# Autodesk Inventor assembly: 02EnsambleJarron
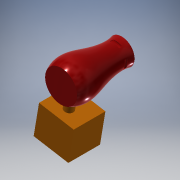
[picture p0: Inventor's stored thumbnail of the model, 180x180]
Saved by Autodesk Inventor 2018 (Build 220112000, 112)
## iProperties
Created: 2020-06-23
Part Number: 02EnsambleJarron
Document SubType Name: Assembly
Designer: Ivan
Author: Ivan
## Documents named in this file (3)
- C:\Users\Ivan\Documents\GitHub\Proyectos980\Modelos3D\02EnsambleJarron.iam
- C:\Users\Ivan\Documents\GitHub\Proyectos980\Modelos3D\02BombaJarron.ipt
- C:\Users\Ivan\Documents\GitHub\Proyectos980\Modelos3D\02Jarron.ipt
## Components (2 placed, 2 different names)
1. 02BombaJarron:1 — Insert:1, Angle:1
2. 02Jarron:1 — Insert:1, Angle:1
## Relationships (2: Insert 1, Angle 1)
- Insert:1 (-5 mm): 02BombaJarron:1 ↔ 02Jarron:1
- Angle:1 (0 deg): 02BombaJarron:1 ↔ 02Jarron:1
